# Autodesk Inventor assembly: Assembly1
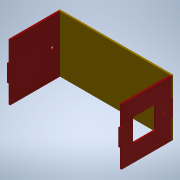
[picture p0: Inventor's stored thumbnail of the model, 180x180]
Saved by Autodesk Inventor 2020 (Build 240168000, 168)
## iProperties
Created: 2020-03-11
Part Number: Assembly1
Document SubType Name: Assembly
Designer: tor16003
Author: tor16003
## Documents named in this file (4)
- C:\Users\joser\OneDrive\Documentos\UVG\2020\Digital 2\Proyecto\Maqueta\Parte alvaro\Proyecto\Assembly1.iam
- C:\Users\joser\OneDrive\Documentos\UVG\2020\Digital 2\Proyecto\Maqueta\Parte alvaro\Proyecto\Part2.ipt
- C:\Users\joser\OneDrive\Documentos\UVG\2020\Digital 2\Proyecto\Maqueta\Parte alvaro\Proyecto\Part3.ipt
- C:\Users\joser\OneDrive\Documentos\UVG\2020\Digital 2\Proyecto\Maqueta\Parte alvaro\Proyecto\Part3 ventilador.ipt
## Components (3 placed, 2 different names)
1. Part2:2 — Coincidencia:1, Coincidencia:2, Coincidencia:3, Coincidencia:4, Coincidencia:5, Coincidencia:6
2. Part3:1 — Coincidencia:1, Coincidencia:2, Coincidencia:3
3. Part3:2 — Coincidencia:4, Coincidencia:5, Coincidencia:6
## Relationships (6: Mate 6)
- Coincidencia:1 [Mate]: Part2:2 ↔ Part3:1
- Coincidencia:2 [Mate]: Part2:2 ↔ Part3:1
- Coincidencia:3 [Mate]: Part2:2 ↔ Part3:1
- Coincidencia:4 [Mate]: Part2:2 ↔ Part3:2
- Coincidencia:5 [Mate]: Part2:2 ↔ Part3:2
- Coincidencia:6 [Mate]: Part2:2 ↔ Part3:2
